# Autodesk Inventor assembly: Housing
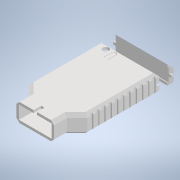
[picture p0: Inventor's stored thumbnail of the model, 180x180]
Saved by Autodesk Inventor 2021 (Build 250183000, 183)
## iProperties
Created: 2021-03-07
Part Number: Housing
Document SubType Name: Assembly
Designer: mista
Author: mista
## Documents named in this file (3)
- C:\Users\mista\Documents\GitHub\node-a\Inventor\Housing.iam
- C:\Users\mista\Documents\GitHub\node-a\Inventor\Cap.ipt
- C:\Users\mista\Documents\GitHub\node-a\Inventor\Shell.ipt
## Components (2 placed, 2 different names)
1. Cap:1 — Mate:1, Flush:1
2. Shell:1 — Mate:1, Flush:1
## Relationships (2: Mate 1, Flush 1)
- Mate:1: Cap:1 ↔ Shell:1
- Flush:1: Cap:1 ↔ Shell:1
